# Autodesk Inventor assembly: SlidingHolder
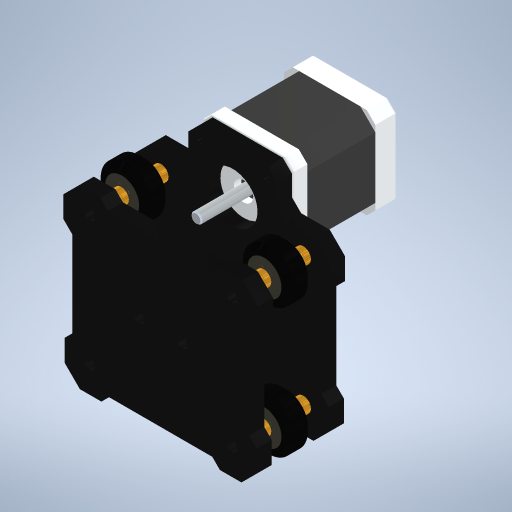
[picture p0: Inventor's stored thumbnail of the model, 512x512]
Saved by Autodesk Inventor 2024.2 (Build 282272000, 272)
## iProperties
Created: 2024-09-03
Part Number: SlidingHolder
Document SubType Name: Assembly
Designer: migue
Author: 1:2
Title: Deslizador Eje Y
## Documents named in this file (6)
- C:\Users\Admin\Documents\GitHub\ManipuladorCartesiano\DiseñoMecánico\Assemblies\SlidingHolder.iam
- C:\Users\Admin\Documents\GitHub\ManipuladorCartesiano\DiseñoMecánico\AcrylicPieces\AxisZ-Carrier1.ipt
- C:\Users\Admin\Documents\GitHub\ManipuladorCartesiano\DiseñoMecánico\AcrylicPieces\AxisZ-Carrier2.ipt
- C:\Users\Admin\Documents\GitHub\ManipuladorCartesiano\DiseñoMecánico\AuxiliarPieces\M5x8-Insert\M5x8-Insert.ipt
- C:\Users\Admin\Documents\GitHub\ManipuladorCartesiano\DiseñoMecánico\AuxiliarPieces\Bearings\625ZZ\NylonPulleyBearing.iam
- C:\Users\Admin\Documents\GitHub\ManipuladorCartesiano\DiseñoMecánico\Motors\NEMA17 [48mm]\NEMA17 [48mm].ipt
## Components (15 placed, 5 different names)
1. AxisZ-Carrier1:1 — Mate:25, Mate:26, Mate:27, Mate:28, Mate:29, Mate:30
2. AxisZ-Carrier2:1 — Mate:17, Mate:18, Mate:19, Mate:20, Mate:21, Mate:22, Mate:23, Mate:24, Mate:25, Mate:26
3. NEMA17 [48mm]:1 — Mate:28, Mate:29, Mate:30
4. M5x8-Insert:2 — Mate:3, Mate:4
5. M5x8-Insert:3 — Mate:1, Mate:2, Mate:19, Mate:20
6. NylonPulleyBearing:3 [sub-assembly] — Mate:1, Mate:2, Mate:3, Mate:4
7. M5x8-Insert:9
8. M5x8-Insert:10 — Mate:23, Mate:24
9. NylonPulleyBearing:5 [sub-assembly]
10. M5x8-Insert:11 — Mate:18, Mate:27
11. M5x8-Insert:12 — Mate:17
12. NylonPulleyBearing:6 [sub-assembly]
13. M5x8-Insert:13 — Mate:22
14. M5x8-Insert:14 — Mate:21
15. NylonPulleyBearing:7 [sub-assembly]
## Relationships (30: Mate 30)
- Mate:1: M5x8-Insert:3 ↔ NylonPulleyBearing:3
- Mate:2: M5x8-Insert:3 ↔ NylonPulleyBearing:3
- Mate:3: M5x8-Insert:2 ↔ NylonPulleyBearing:3
- Mate:4: M5x8-Insert:2 ↔ NylonPulleyBearing:3
- [Mate]: M5x8-Insert:10 ↔ NylonPulleyBearing:5
- [Mate]: M5x8-Insert:10 ↔ NylonPulleyBearing:5
- [Mate]: M5x8-Insert:9 ↔ NylonPulleyBearing:5
- [Mate]: M5x8-Insert:9 ↔ NylonPulleyBearing:5
- [Mate]: M5x8-Insert:12 ↔ NylonPulleyBearing:6
- [Mate]: M5x8-Insert:12 ↔ NylonPulleyBearing:6
- [Mate]: M5x8-Insert:11 ↔ NylonPulleyBearing:6
- [Mate]: M5x8-Insert:11 ↔ NylonPulleyBearing:6
- [Mate]: M5x8-Insert:14 ↔ NylonPulleyBearing:7
- [Mate]: M5x8-Insert:14 ↔ NylonPulleyBearing:7
- [Mate]: M5x8-Insert:13 ↔ NylonPulleyBearing:7
- [Mate]: M5x8-Insert:13 ↔ NylonPulleyBearing:7
- Mate:17: AxisZ-Carrier2:1 ↔ M5x8-Insert:12
- Mate:18: AxisZ-Carrier2:1 ↔ M5x8-Insert:11
- Mate:19: AxisZ-Carrier2:1 ↔ M5x8-Insert:3
- Mate:20: AxisZ-Carrier2:1 ↔ M5x8-Insert:3
- Mate:21: AxisZ-Carrier2:1 ↔ M5x8-Insert:14
- Mate:22: AxisZ-Carrier2:1 ↔ M5x8-Insert:13
- Mate:23: AxisZ-Carrier2:1 ↔ M5x8-Insert:10
- Mate:24: AxisZ-Carrier2:1 ↔ M5x8-Insert:10
- Mate:25: AxisZ-Carrier1:1 ↔ AxisZ-Carrier2:1
- Mate:26: AxisZ-Carrier1:1 ↔ AxisZ-Carrier2:1
- Mate:27: AxisZ-Carrier1:1 ↔ M5x8-Insert:11
- Mate:28: AxisZ-Carrier1:1 ↔ NEMA17 [48mm]:1
- Mate:29: AxisZ-Carrier1:1 ↔ NEMA17 [48mm]:1
- Mate:30: AxisZ-Carrier1:1 ↔ NEMA17 [48mm]:1
## Named parameters: d4_d0 = 0 mm, d5_d1 = 0 mm, d6_d2 = 0 mm, d7_d3 = 0 mm, d8_d0 = 0 mm, d9_d1 = 0 mm, d10_d2 = 0 mm, d11_d3 = 0 mm, d12_d0 = 0 mm, d13_d1 = 0 mm, d14_d2 = 0 mm, d15_d3 = 0 mm
